# Autodesk Inventor assembly: Assembly1
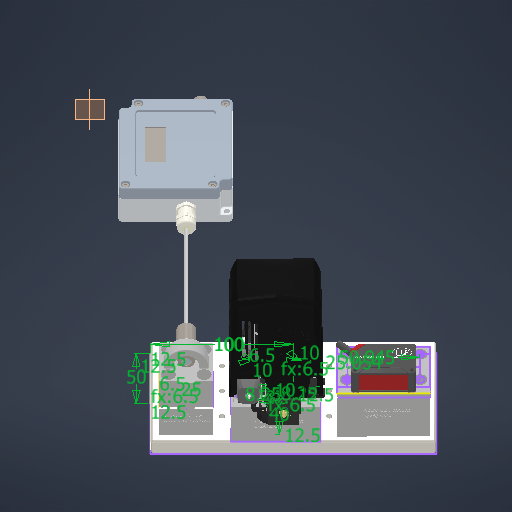
[picture p0: Inventor's stored thumbnail of the model, 512x512]
Saved by Autodesk Inventor 2027 (Build 310192060, 192F)
## iProperties
Created: 2026-05-22
Part Number: Assembly1
Document SubType Name: Assembly
Designer: jacob
Author: jacob
## Documents named in this file (9)
- C:\Users\jacob\Documents\Autodesk\Inventor 2027\mount_proj_v2\Assembly.iam
- C:\Users\jacob\Documents\Autodesk\Inventor 2027\mount_proj_v2\ILD1x20-500\ILD1x20-500.ipt
- C:\Users\jacob\Documents\Autodesk\Inventor 2027\mount_proj_v2\Mount.ipt
- C:\Users\jacob\Documents\Autodesk\Inventor 2027\mount_proj_v2\thermoMETER UC\thermoMETER UC.ipt
- C:\Users\jacob\Documents\Autodesk\Inventor 2027\mount_proj_v2\optoNCDT_mount.ipt
- C:\Users\jacob\Documents\Autodesk\Inventor 2027\mount_proj_v2\thermoMETER_mount.ipt
- C:\Users\jacob\Documents\Autodesk\Inventor 2027\mount_proj_v2\tm_top.ipt
- C:\Users\jacob\Documents\Autodesk\Inventor 2027\mount_proj_v2\Printer_head_mount.ipt
- C:\Users\jacob\Documents\Autodesk\Inventor 2027\mount_proj_v2\ender-3v3-se-head-cad\cad of ender 3v3 se head\cad of ender 3v3 se head.ipt
## Components (8 placed, 8 different names)
1. Printer_head_mount:1 — Flush:5, Flush:6
2. bottom — Mate:4, Mate:7
3. tm_top:1 — Mate:6
4. tm_bottom — Mate:5, Mate:6
5. thermoMETER UC:1
6. ILD1x20-500:1 — Mate:7
7. cad of ender 3v3 se head:1
8. Mount:1 — Flush:5, Flush:6, Mate:4, Mate:5
## Relationships (6: Mate 4, Flush 2)
- Flush:5: Printer_head_mount:1 ↔ Mount:1
- Flush:6: Printer_head_mount:1 ↔ Mount:1
- Mate:4: bottom ↔ Mount:1
- Mate:5: tm_bottom ↔ Mount:1
- Mate:6: tm_top:1 ↔ tm_bottom
- Mate:7: bottom ↔ ILD1x20-500:1
